# Autodesk Inventor assembly: full
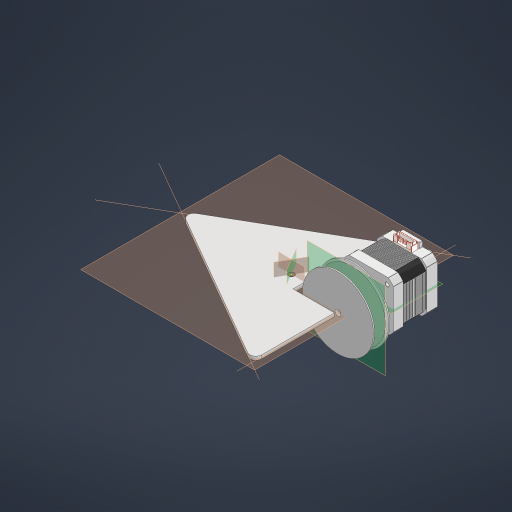
[picture p0: Inventor's stored thumbnail of the model, 512x512]
Saved by Autodesk Inventor 2024 (Build 280153000, 153)
## iProperties
Created: 2026-03-23
Part Number: full
Document SubType Name: Assembly
Designer: schar
Author: schar
## Documents named in this file (4)
- C:\Users\schar\Desktop\FloatingFace\models\full.iam
- C:\Users\schar\Desktop\FloatingFace\models\baseplate.ipt
- C:\Users\schar\Desktop\FloatingFace\models\spool.ipt
- C:\Users\schar\Desktop\FloatingFace\models\17HS4401S_Stepper_Motor\17HS4401S_Stepper_Motor.iam
## Components (3 placed, 3 different names)
1. baseplate:1 — Mate:1, Mate:2, Mate:3
2. spool:1 — Mate:1, Mate:2, Mate:4, Mate:5
3. 17HS4401S_Stepper_Motor:1 [sub-assembly] — Mate:3, Mate:4, Mate:5
## Relationships (5: Mate 5)
- Mate:1: baseplate:1 ↔ spool:1
- Mate:2: baseplate:1 ↔ spool:1
- Mate:3: baseplate:1 ↔ 17HS4401S_Stepper_Motor:1
- Mate:4: spool:1 ↔ 17HS4401S_Stepper_Motor:1
- Mate:5: spool:1 ↔ 17HS4401S_Stepper_Motor:1
